# Autodesk Inventor assembly: голова - сборка
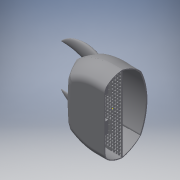
[picture p0: Inventor's stored thumbnail of the model, 180x180]
Saved by Autodesk Inventor 2019 (Build 230136000, 136)
## iProperties
Created: 2019-09-05
Part Number: голова - сборка
Material: Типовые
Document SubType Name: Assembly
Designer: Iliga
Author: Iliga
## Documents named in this file (5)
- C:\Users\Iliga\Desktop\робот\голова - сборка.iam
- C:\Users\Iliga\Desktop\робот\голова.ipt
- C:\Users\Iliga\Desktop\робот\двигатель.ipt
- C:\Users\Iliga\Desktop\робот\хелицера-левая.ipt
- C:\Users\Iliga\Desktop\робот\хелицера-правая.ipt
## Components (5 placed, 3 different names)
1. голова:1 — Совмещение:1, Совмещение:2, Совмещение:4, Совмещение:5, Совмещение:11, Совмещение:12
2. двигатель:1 — Совмещение:1, Совмещение:2, Совмещение:7, Совмещение:8, Совмещение:11
3. двигатель:2 — Совмещение:4, Совмещение:5, Совмещение:10, Совмещение:12, Совмещение:13
4. хелицера:1 — Совмещение:7, Совмещение:8
5. хелицера:2 — Совмещение:10, Совмещение:13
## Relationships (10: Mate 10)
- Совмещение:1 [Mate]: голова:1 ↔ двигатель:1
- Совмещение:2 [Mate]: голова:1 ↔ двигатель:1
- Совмещение:4 [Mate]: голова:1 ↔ двигатель:2
- Совмещение:5 [Mate]: голова:1 ↔ двигатель:2
- Совмещение:7 [Mate]: двигатель:1 ↔ хелицера:1
- Совмещение:8 [Mate]: двигатель:1 ↔ хелицера:1
- Совмещение:10 [Mate]: двигатель:2 ↔ хелицера:2
- Совмещение:11 [Mate]: голова:1 ↔ двигатель:1
- Совмещение:12 [Mate]: голова:1 ↔ двигатель:2
- Совмещение:13 [Mate]: двигатель:2 ↔ хелицера:2
